# Autodesk Inventor assembly: LegGroinUnit
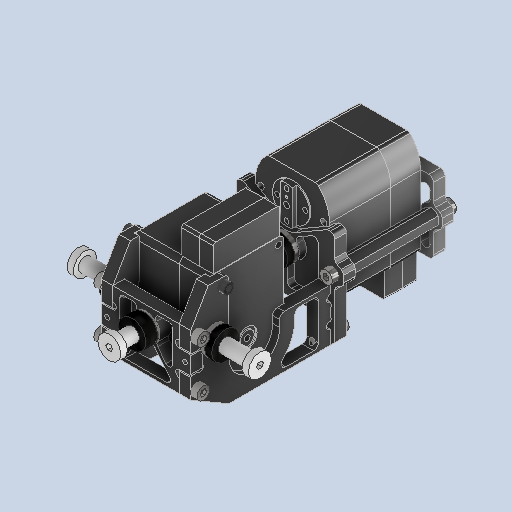
[picture p0: Inventor's stored thumbnail of the model, 512x512]
Saved by Autodesk Inventor 2024.2 (Build 282272000, 272)
## iProperties
Created: 2024-01-08
Part Number: LegGroinUnit
Document SubType Name: Assembly
Designer: Masato Kubotera
Mass: 305.382 g
Surface Area: 472.823 cm^2
Volume: 134.011 cm^3
Density: 2.27879 g/cm^3
Author: Masato Kubotera
## Documents named in this file (5)
- C:\Users\masato\OneDrive - Chiba Institute of Technology\CIT Brains\RoboCup2024\Mechanic\SUSTAINA-OP2-DEV\NativeFiles\Boby\LowerLimb\Legs\LegBases\LegGroinUnit.iam
- C:\Users\masato\OneDrive - Chiba Institute of Technology\CIT Brains\RoboCup2024\Mechanic\SUSTAINA-OP2-DEV\NativeFiles\Boby\COTS\Actuators\PMX-SCR-5203HV.ipt
- C:\Users\masato\OneDrive - Chiba Institute of Technology\CIT Brains\RoboCup2024\Mechanic\SUSTAINA-OP2-DEV\NativeFiles\Boby\COTS\Screws\CapScrew\FC-2615EB.ipt
- C:\Users\masato\OneDrive - Chiba Institute of Technology\CIT Brains\RoboCup2024\Mechanic\SUSTAINA-OP2-DEV\NativeFiles\Boby\COTS\Screws\CapScrew\FC-2620EB.ipt
- C:\Users\masato\OneDrive - Chiba Institute of Technology\CIT Brains\RoboCup2024\Mechanic\SUSTAINA-OP2-DEV\NativeFiles\Boby\LowerLimb\Legs\LegBases\LegGroinUnitBasis.iam
## Components (4 placed, 4 different names)
1. LegGroinUnitBasis:1 [sub-assembly] — Flush:1, Flush:2, Flush:3, Insert:1, Insert:2, Insert:3, Insert:4
2. PMX-SCR-5203HV:1 — Insert:1, Insert:2
3. FC-2615EB:1 — Insert:3
4. FC-2620EB:1 — Insert:4
## Relationships (7: Insert 4, Flush 3)
- Flush:1: LegGroinUnitBasis:1
- Flush:2: LegGroinUnitBasis:1
- Flush:3: LegGroinUnitBasis:1
- Insert:1: LegGroinUnitBasis:1 ↔ PMX-SCR-5203HV:1
- Insert:2: LegGroinUnitBasis:1 ↔ PMX-SCR-5203HV:1
- Insert:3: LegGroinUnitBasis:1 ↔ FC-2615EB:1
- Insert:4: LegGroinUnitBasis:1 ↔ FC-2620EB:1
